# Autodesk Inventor assembly: cycloid_top_bottom_assy
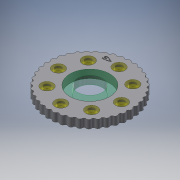
[picture p0: Inventor's stored thumbnail of the model, 180x180]
Saved by Autodesk Inventor 2019.4 (Build 234330000, 330)
## iProperties
Created: 2019-08-28
Part Number: cycloid_top_bottom_assy
Document SubType Name: Assembly
Designer: cdi
Author: cdi
## Documents named in this file (4)
- D:\SynologyDrive\workspace_inventor\2019_06_19.MT4008_actuator\cycloid_gear_design_v2\cycloid_top_bottom_assy.iam
- D:\SynologyDrive\workspace_inventor\2019_06_19.MT4008_actuator\cycloid_gear_design_v2\cycloid_top_bottom.ipt
- D:\SynologyDrive\workspace_inventor\2019_06_19.MT4008_actuator\cycloid_gear_design_v2\bearing_4_7_2.5.ipt
- D:\SynologyDrive\workspace_inventor\2019_06_19.MT4008_actuator\cycloid_gear_design_v2\bearing_15_24_5.ipt
## Components (18 placed, 3 different names)
1. cycloid_top_bottom:1 — Mate:3, Mate:4, Mate:5, Mate:6, Flush:1, Flush:2, Mate:7, Flush:3
2. bearing_15_24_5:1 — Mate:7, Flush:3
3. bearing_4_7_2.5:1 — Mate:5, Flush:2
4. bearing_4_7_2.5:2 — Mate:6, Flush:1
5. bearing_4_7_2.5:3
6. bearing_4_7_2.5:4
7. bearing_4_7_2.5:5
8. bearing_4_7_2.5:6
9. bearing_4_7_2.5:7
10. bearing_4_7_2.5:8
11. bearing_4_7_2.5:9
12. bearing_4_7_2.5:10
13. bearing_4_7_2.5:11
14. bearing_4_7_2.5:12
15. bearing_4_7_2.5:13
16. bearing_4_7_2.5:14
17. bearing_4_7_2.5:15
18. bearing_4_7_2.5:16
## Component patterns: (8 elements, first: bearing_4_7_2.5:1 + bearing_4_7_2.5:2)
## Relationships (8: Mate 5, Flush 3)
- Mate:3: cycloid_top_bottom:1
- Mate:4: cycloid_top_bottom:1
- Mate:5: cycloid_top_bottom:1 ↔ bearing_4_7_2.5:1
- Mate:6: cycloid_top_bottom:1 ↔ bearing_4_7_2.5:2
- Flush:1: cycloid_top_bottom:1 ↔ bearing_4_7_2.5:2
- Flush:2: cycloid_top_bottom:1 ↔ bearing_4_7_2.5:1
- Mate:7: cycloid_top_bottom:1 ↔ bearing_15_24_5:1
- Flush:3: cycloid_top_bottom:1 ↔ bearing_15_24_5:1
